# Autodesk Inventor assembly: WCD
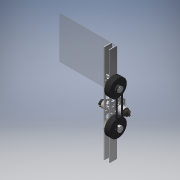
[picture p0: Inventor's stored thumbnail of the model, 180x180]
Saved by Autodesk Inventor 2019.4 (Build 234330000, 330)
## iProperties
Created: 2019-12-06
Part Number: WCD
Document SubType Name: Assembly
Designer: Mark
Mass: 6451.53 g
Surface Area: 5888.72 cm^2
Volume: 2850.82 cm^3
Density: 2.26305 g/cm^3
Author: Mark
## Documents named in this file (16)
- C:\Users\Mark\Desktop\7738 Helion Engineering\7738-CAD-prep\WCD\WCD.iam
- C:\Users\Mark\Desktop\7738 Helion Engineering\7738-CAD-prep\WCD\Cheese.ipt
- C:\Users\Mark\Desktop\7738 Helion Engineering\7738-CAD-prep\Swerve Module\Falcon_500_Powered_by_Talon_FX_217-6515.iam
- C:\Users\Mark\Desktop\7738 Helion Engineering\7738-CAD-prep\WCD\F6902.ipt
- C:\Users\Mark\Desktop\7738 Helion Engineering\7738-CAD-prep\WCD\F63800zz.ipt
- C:\Users\Mark\Desktop\7738 Helion Engineering\7738-CAD-prep\WCD\WCD\Design Accelerator\Spur Gears1.iam
- C:\Users\Mark\Desktop\7738 Helion Engineering\7738-CAD-prep\WCD\WCD\Design Accelerator\Spur Gears2.iam
- C:\Users\Mark\Desktop\7738 Helion Engineering\7738-CAD-prep\WCD\WCD\Design Accelerator\Spur Gears3.iam
- C:\Users\Mark\Desktop\7738 Helion Engineering\7738-CAD-prep\WCD\Spacer.ipt
- C:\Users\Mark\Desktop\7738 Helion Engineering\7738-CAD-prep\WCD\Wheel.ipt
- C:\Users\Mark\Desktop\7738 Helion Engineering\7738-CAD-prep\WCD\30 T Pulley.ipt
- C:\Users\Mark\Desktop\7738 Helion Engineering\7738-CAD-prep\WCD\Belt 750.ipt
- C:\Users\Mark\Desktop\7738 Helion Engineering\7738-CAD-prep\WCD\WCD\Design Accelerator\Shaft1.iam
- C:\Users\Mark\Desktop\7738 Helion Engineering\7738-CAD-prep\WCD\WCD\Design Accelerator\Shaft3.iam
- C:\Users\Mark\Desktop\7738 Helion Engineering\7738-CAD-prep\WCD\WCD\Design Accelerator\Shaft4.iam
- C:\Users\Mark\Desktop\7738 Helion Engineering\7738-CAD-prep\WCD\Width plate.ipt
## Components (34 placed, 11 different names)
1. Cheese:2 — Mate:2, Mate:3, Mate:4, Mate:6, Mate:7, Mate:8, Mate:9, Mate:12, Mate:13, Mate:18, Mate:19, Mate:20, Mate:21, Mate:22, Mate:23, Mate:25, Mate:26, Mate:28, Mate:29, Mate:30, Mate:31, Mate:32, Mate:37, Mate:40, Mate:42, Mate:43, Mate:64, Mate:65, Mate:66, Mate:67, Mate:71, Mate:73
2. Cheese:1 — Mate:1, Mate:2, Mate:3, Mate:4, Mate:5, Mate:10, Mate:11, Mate:14, Mate:15, Mate:16, Mate:17, Mate:35, Mate:38, Mate:39, Mate:41, Mate:44, Mate:45, Mate:46, Mate:48, Mate:50, Mate:61, Mate:63, Mate:68, Mate:69, Mate:70, Mate:72, Flush:1
3. Wheel:1 — Mate:47, Mate:48, Mate:51, Mate:52
4. Wheel:2 — Mate:49, Mate:50, Mate:53, Mate:54, Mate:57
5. Shaft:1 [sub-assembly] — Mate:58, Mate:59
6. Shaft:2 [sub-assembly] — Mate:60, Mate:61
7. Shaft:3 [sub-assembly] — Mate:62, Mate:63
8. Width plate:1 — Mate:72, Flush:1, Mate:73
9. F63800zz:2 — Mate:18, Mate:19
10. F6902:3 — Mate:14, Mate:15, Mate:49, Mate:60
11. F63800zz:1 — Mate:16, Mate:17, Mate:24, Mate:58, Mate:59
12. F6902:4 — Mate:20, Mate:21
13. F6902:2 — Mate:12, Mate:13
14. F6902:1 — Mate:10, Mate:11, Mate:47, Mate:62
15. Falcon_500_Powered_by_Talon_FX_217-6515:3 [sub-assembly] — Mate:6, Mate:7
16. Falcon_500_Powered_by_Talon_FX_217-6515:2 [sub-assembly] — Mate:1, Mate:5
17. Falcon_500_Powered_by_Talon_FX_217-6515:1 [sub-assembly] — Mate:8, Mate:9
18. Belt 750:1 — Mate:55, Mate:56, Mate:57
19. 30 T Pulley:1 — Mate:51, Mate:52, Mate:55
20. 30 T Pulley:2 — Mate:53, Mate:54, Mate:56
21. Spur Gears:1 [sub-assembly] — Mate:22, Mate:23, Mate:24, Mate:27
22. Spur Gears:2 [sub-assembly] — Mate:25, Mate:26, Mate:27
23. Spur Gears:3 [sub-assembly] — Mate:28, Mate:29
24. Spur Gears:4 [sub-assembly] — Mate:30, Mate:31
25. Spacer:10 — Mate:70, Mate:71
26. Spacer:7 — Mate:64, Mate:65
27. Spacer:8 — Mate:66, Mate:67
28. Spacer:9 — Mate:68, Mate:69
29. Spacer:2 — Mate:35, Mate:41
30. Spacer:3 — Mate:37, Mate:40
31. Spacer:4 — Mate:38, Mate:39
32. Spacer:5 — Mate:43, Mate:44
33. Spacer:6 — Mate:45, Mate:46
34. Spacer:1 — Mate:32, Mate:42
## Relationships (71: Mate 70, Flush 1)
- Mate:1: Cheese:1 ↔ Falcon_500_Powered_by_Talon_FX_217-6515:2
- Mate:2 (37 mm): Cheese:2 ↔ Cheese:1
- Mate:3: Cheese:2 ↔ Cheese:1
- Mate:4: Cheese:2 ↔ Cheese:1
- Mate:5: Cheese:1 ↔ Falcon_500_Powered_by_Talon_FX_217-6515:2
- Mate:6: Cheese:2 ↔ Falcon_500_Powered_by_Talon_FX_217-6515:3
- Mate:7: Cheese:2 ↔ Falcon_500_Powered_by_Talon_FX_217-6515:3
- Mate:8: Cheese:2 ↔ Falcon_500_Powered_by_Talon_FX_217-6515:1
- Mate:9: Cheese:2 ↔ Falcon_500_Powered_by_Talon_FX_217-6515:1
- Mate:10: Cheese:1 ↔ F6902:1
- Mate:11: Cheese:1 ↔ F6902:1
- Mate:12: Cheese:2 ↔ F6902:2
- Mate:13: Cheese:2 ↔ F6902:2
- Mate:14: Cheese:1 ↔ F6902:3
- Mate:15: Cheese:1 ↔ F6902:3
- Mate:16: Cheese:1 ↔ F63800zz:1
- Mate:17: Cheese:1 ↔ F63800zz:1
- Mate:18: Cheese:2 ↔ F63800zz:2
- Mate:19: Cheese:2 ↔ F63800zz:2
- Mate:20: Cheese:2 ↔ F6902:4
- Mate:21: Cheese:2 ↔ F6902:4
- Mate:22: Cheese:2 ↔ Spur Gears:1
- Mate:23: Cheese:2 ↔ Spur Gears:1
- Mate:24 (2.65 mm): F63800zz:1 ↔ Spur Gears:1
- Mate:25: Cheese:2 ↔ Spur Gears:2
- Mate:26: Cheese:2 ↔ Spur Gears:2
- Mate:27 (1 mm): Spur Gears:1 ↔ Spur Gears:2
- Mate:28: Cheese:2 ↔ Spur Gears:3
- Mate:29 (4.315 mm): Cheese:2 ↔ Spur Gears:3
- Mate:30: Cheese:2 ↔ Spur Gears:4
- Mate:31 (4.315 mm): Cheese:2 ↔ Spur Gears:4
- Mate:32: Cheese:2 ↔ Spacer:1
- Mate:35: Cheese:1 ↔ Spacer:2
- Mate:37: Cheese:2 ↔ Spacer:3
- Mate:38: Cheese:1 ↔ Spacer:4
- Mate:39: Cheese:1 ↔ Spacer:4
- Mate:40: Cheese:2 ↔ Spacer:3
- Mate:41: Cheese:1 ↔ Spacer:2
- Mate:42: Cheese:2 ↔ Spacer:1
- Mate:43: Cheese:2 ↔ Spacer:5
- Mate:44: Cheese:1 ↔ Spacer:5
- Mate:45: Cheese:1 ↔ Spacer:6
- Mate:46: Cheese:1 ↔ Spacer:6
- Mate:47: Wheel:1 ↔ F6902:1
- Mate:48 (4 mm): Cheese:1 ↔ Wheel:1
- Mate:49: Wheel:2 ↔ F6902:3
- Mate:50 (4 mm): Cheese:1 ↔ Wheel:2
- Mate:51: Wheel:1 ↔ 30 T Pulley:1
- Mate:52: Wheel:1 ↔ 30 T Pulley:1
- Mate:53: Wheel:2 ↔ 30 T Pulley:2
- Mate:54: Wheel:2 ↔ 30 T Pulley:2
- Mate:55: Belt 750:1 ↔ 30 T Pulley:1
- Mate:56: Belt 750:1 ↔ 30 T Pulley:2
- Mate:57 (3 mm): Wheel:2 ↔ Belt 750:1
- Mate:58: Shaft:1 ↔ F63800zz:1
- Mate:59: Shaft:1 ↔ F63800zz:1
- Mate:60: Shaft:2 ↔ F6902:3
- Mate:61: Cheese:1 ↔ Shaft:2
- Mate:62: Shaft:3 ↔ F6902:1
- Mate:63: Cheese:1 ↔ Shaft:3
- Mate:64: Cheese:2 ↔ Spacer:7
- Mate:65: Cheese:2 ↔ Spacer:7
- Mate:66: Cheese:2 ↔ Spacer:8
- Mate:67: Cheese:2 ↔ Spacer:8
- Mate:68: Cheese:1 ↔ Spacer:9
- Mate:69: Cheese:1 ↔ Spacer:9
- Mate:70: Cheese:1 ↔ Spacer:10
- Mate:71: Cheese:2 ↔ Spacer:10
- Mate:72: Cheese:1 ↔ Width plate:1
- Flush:1: Cheese:1 ↔ Width plate:1
- Mate:73: Cheese:2 ↔ Width plate:1
